# Autodesk Inventor assembly: Assembly1
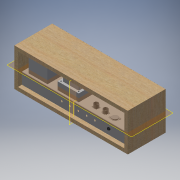
[picture p0: Inventor's stored thumbnail of the model, 180x180]
Saved by Autodesk Inventor 2016 (Build 200138000, 138)
## iProperties
Created: 2015-10-14
Part Number: Assembly1
Document SubType Name: Assembly
Designer: jeremyhale
Author: jeremyhale
## Documents named in this file (16)
- \\psf\Home\Documents\Poorhouse\Amps\p0001\Assembly1.iam
- \\psf\Home\Documents\Poorhouse\Amps\p0001\chassis.ipt
- \\psf\Home\Documents\Poorhouse\Amps\p0001\tube socket 8 pin.ipt
- \\psf\Home\Documents\Poorhouse\Amps\p0001\tube socket 9 pin.ipt
- \\psf\Home\Documents\Poorhouse\Amps\p0001\xmfr power.ipt
- \\psf\Home\Documents\Poorhouse\Amps\p0001\xmfr output.ipt
- \\psf\Home\Documents\Inventor\Content Center Files\R2016\en-US\AS 1427(08)\AS 1427 - M3 x 5(6) I.ipt
- \\psf\Home\Documents\Inventor\Content Center Files\R2016\en-US\AS 1474(1)\AS 1474 - M2.5(1).ipt
- \\psf\Home\Documents\Inventor\Content Center Files\R2016\en-US\AS 1474(1)\AS 1474 - M3.5(1).ipt
- \\psf\Home\Documents\Inventor\Content Center Files\R2016\en-US\AS 1474(1)\AS 1474 - M3(1).ipt
- \\psf\Home\Documents\Poorhouse\Amps\p0001\cabinet.ipt
- \\psf\Home\Documents\Poorhouse\Amps\p0001\iec320_703W-00_04.ipt
- \\psf\Home\Documents\Inventor\Content Center Files\R2016\en-US\AS 1427(07)\AS 1427 - M3 x 10(6) II.ipt
- \\psf\Home\Downloads\switch-toggle.snapshot.2\Toggle_Large_A\Toggle Large A.ipt
- \\psf\Home\Downloads\audio-jack-model-2-1.snapshot.2\AUDIO JACK 2.ipt
- \\psf\Home\Downloads\audio-jack-model-2-1.snapshot.2\AUDIO JACK 2_CPY.ipt
## Components (58 placed, 15 different names)
1. chassis:1 — Rotational:1, Rotational:2, Rotational:3, Rotational:4, Rotational:5, Rotational:6, Rotational:7, Rotational:8, Rotational:9, Rotational:10, Mate:4, Insert:20, Insert:21, Insert:22, Insert:23, Insert:24, Insert:25, Insert:26, Insert:27, Insert:28, Insert:29, Insert:30, Insert:31, Insert:32, Insert:33, Insert:34, Insert:35, Insert:36, Insert:37, Flush:1, Mate:5, Flush:2, Rotational:11, Rotational:12, Mate:11, Mate:13, Rigid:14, Rigid:15, Rigid:16
2. tube socket 8 pin:7 — Rotational:3, Rotational:4, Insert:13, Insert:14
3. xmfr power:1 — Rotational:7, Rotational:8
4. xmfr output:1 — Rotational:9, Rotational:10
5. cabinet:1 — Flush:1, Mate:5, Flush:2
6. iec320_703W-00_04:1 — Rotational:11, Rotational:12, Mate:6, Mate:7
7. AS 1427 Z - Metric M3 x 10:2 — Mate:6, Mate:10
8. AS 1427 Z - Metric M3 x 10:1 — Mate:7, Mate:12
9. AS 1474 - Metric M3:5 — Mate:10, Mate:11
10. AS 1474 - Metric M3:6 — Mate:12, Mate:13
11. Toggle Large A:1 — Rigid:14
12. AUDIO JACK 2:1 — Rigid:15
13. AUDIO JACK 2_CPY:1 — Rigid:16
14. AS 1427 Z - Metric M3 x 5:1 — Insert:1, Mate:3
15. AS 1427 Z - Metric M3 x 5:2 — Insert:2
16. AS 1427 Z - Metric M3 x 5:3 — Insert:3
17. AS 1427 Z - Metric M3 x 5:4 — Insert:4
18. AS 1427 Z - Metric M3 x 5:5 — Insert:5
19. AS 1427 Z - Metric M3 x 5:6 — Insert:6
20. AS 1427 Z - Metric M3 x 5:7 — Insert:7
21. AS 1427 Z - Metric M3 x 5:8 — Insert:8
22. AS 1427 Z - Metric M3 x 5:9 — Insert:9
23. AS 1427 Z - Metric M3 x 5:10 — Insert:10
24. AS 1427 Z - Metric M3 x 5:11 — Insert:11
25. AS 1427 Z - Metric M3 x 5:12 — Insert:12
26. AS 1427 Z - Metric M3 x 5:13 — Insert:13
27. AS 1427 Z - Metric M3 x 5:14 — Insert:14
28. AS 1427 Z - Metric M3 x 5:15 — Insert:15
29. AS 1427 Z - Metric M3 x 5:16 — Insert:16
30. AS 1427 Z - Metric M3 x 5:17 — Insert:17
31. AS 1427 Z - Metric M3 x 5:18 — Insert:18
32. AS 1474 - Metric M2.5:1 — Mate:3, Mate:4
33. AS 1474 - Metric M3.5:1 — Insert:20
34. AS 1474 - Metric M3.5:2 — Insert:21
35. AS 1474 - Metric M3.5:3 — Insert:22
36. AS 1474 - Metric M3.5:4 — Insert:23
37. AS 1474 - Metric M3.5:5 — Insert:24
38. AS 1474 - Metric M3.5:6 — Insert:25
39. AS 1474 - Metric M3.5:7 — Insert:26
40. AS 1474 - Metric M3.5:8 — Insert:27
41. AS 1474 - Metric M3.5:9 — Insert:28
42. AS 1474 - Metric M3.5:10 — Insert:29
43. AS 1474 - Metric M3.5:11 — Insert:30
44. AS 1474 - Metric M3.5:12 — Insert:31
45. AS 1474 - Metric M3.5:13 — Insert:32
46. AS 1474 - Metric M3.5:14 — Insert:33
47. AS 1474 - Metric M3:1 — Insert:34
48. AS 1474 - Metric M3:2 — Insert:35
49. AS 1474 - Metric M3:3 — Insert:36
50. AS 1474 - Metric M3:4 — Insert:37
51. tube socket 8 pin:1 — Rotational:1, Rotational:2, Insert:1, Insert:2
52. tube socket 8 pin:2 — Insert:3, Insert:4
53. tube socket 8 pin:3 — Insert:5, Insert:6
54. tube socket 8 pin:4 — Insert:7, Insert:8
55. tube socket 8 pin:5 — Insert:15, Insert:16
56. tube socket 8 pin:6 — Insert:17, Insert:18
57. tube socket 9 pin:1 — Rotational:5, Rotational:6, Insert:9, Insert:10
58. tube socket 9 pin:2 — Insert:11, Insert:12
## Component patterns: Big Tube Sockets (6 elements), (2 elements, first: tube socket 9 pin:1)
## Relationships (62: Insert 36, RevoluteJoint 12, Mate 9, WeldJoint 3, Flush 2)
- Rotational:1 [RevoluteJoint]: chassis:1 ↔ tube socket 8 pin:1
- Rotational:2 [RevoluteJoint]: chassis:1 ↔ tube socket 8 pin:1
- Rotational:3 [RevoluteJoint]: chassis:1 ↔ tube socket 8 pin:7
- Rotational:4 [RevoluteJoint]: chassis:1 ↔ tube socket 8 pin:7
- Rotational:5 [RevoluteJoint]: chassis:1 ↔ tube socket 9 pin:1
- Rotational:6 [RevoluteJoint]: chassis:1 ↔ tube socket 9 pin:1
- Rotational:7 [RevoluteJoint]: chassis:1 ↔ xmfr power:1
- Rotational:8 [RevoluteJoint]: chassis:1 ↔ xmfr power:1
- Rotational:9 [RevoluteJoint]: chassis:1 ↔ xmfr output:1
- Rotational:10 [RevoluteJoint]: chassis:1 ↔ xmfr output:1
- Insert:1: AS 1427 Z - Metric M3 x 5:1 ↔ tube socket 8 pin:1
- Insert:2: AS 1427 Z - Metric M3 x 5:2 ↔ tube socket 8 pin:1
- Insert:3: AS 1427 Z - Metric M3 x 5:3 ↔ tube socket 8 pin:2
- Insert:4: AS 1427 Z - Metric M3 x 5:4 ↔ tube socket 8 pin:2
- Insert:5: AS 1427 Z - Metric M3 x 5:5 ↔ tube socket 8 pin:3
- Insert:6: AS 1427 Z - Metric M3 x 5:6 ↔ tube socket 8 pin:3
- Insert:7: AS 1427 Z - Metric M3 x 5:7 ↔ tube socket 8 pin:4
- Insert:8: AS 1427 Z - Metric M3 x 5:8 ↔ tube socket 8 pin:4
- Insert:9: AS 1427 Z - Metric M3 x 5:9 ↔ tube socket 9 pin:1
- Insert:10: AS 1427 Z - Metric M3 x 5:10 ↔ tube socket 9 pin:1
- Insert:11: AS 1427 Z - Metric M3 x 5:11 ↔ tube socket 9 pin:2
- Insert:12: AS 1427 Z - Metric M3 x 5:12 ↔ tube socket 9 pin:2
- Insert:13: tube socket 8 pin:7 ↔ AS 1427 Z - Metric M3 x 5:13
- Insert:14: tube socket 8 pin:7 ↔ AS 1427 Z - Metric M3 x 5:14
- Insert:15: AS 1427 Z - Metric M3 x 5:15 ↔ tube socket 8 pin:5
- Insert:16: AS 1427 Z - Metric M3 x 5:16 ↔ tube socket 8 pin:5
- Insert:17: AS 1427 Z - Metric M3 x 5:17 ↔ tube socket 8 pin:6
- Insert:18: AS 1427 Z - Metric M3 x 5:18 ↔ tube socket 8 pin:6
- Mate:3: AS 1427 Z - Metric M3 x 5:1 ↔ AS 1474 - Metric M2.5:1
- Mate:4: chassis:1 ↔ AS 1474 - Metric M2.5:1
- Insert:20: chassis:1 ↔ AS 1474 - Metric M3.5:1
- Insert:21: chassis:1 ↔ AS 1474 - Metric M3.5:2
- Insert:22: chassis:1 ↔ AS 1474 - Metric M3.5:3
- Insert:23: chassis:1 ↔ AS 1474 - Metric M3.5:4
- Insert:24: chassis:1 ↔ AS 1474 - Metric M3.5:5
- Insert:25: chassis:1 ↔ AS 1474 - Metric M3.5:6
- Insert:26: chassis:1 ↔ AS 1474 - Metric M3.5:7
- Insert:27: chassis:1 ↔ AS 1474 - Metric M3.5:8
- Insert:28: chassis:1 ↔ AS 1474 - Metric M3.5:9
- Insert:29: chassis:1 ↔ AS 1474 - Metric M3.5:10
- Insert:30: chassis:1 ↔ AS 1474 - Metric M3.5:11
- Insert:31: chassis:1 ↔ AS 1474 - Metric M3.5:12
- Insert:32: chassis:1 ↔ AS 1474 - Metric M3.5:13
- Insert:33: chassis:1 ↔ AS 1474 - Metric M3.5:14
- Insert:34: chassis:1 ↔ AS 1474 - Metric M3:1
- Insert:35: chassis:1 ↔ AS 1474 - Metric M3:2
- Insert:36: chassis:1 ↔ AS 1474 - Metric M3:3
- Insert:37: chassis:1 ↔ AS 1474 - Metric M3:4
- Flush:1: chassis:1 ↔ cabinet:1
- Mate:5: chassis:1 ↔ cabinet:1
- Flush:2 (-19.05 mm): chassis:1 ↔ cabinet:1
- Rotational:11 [RevoluteJoint]: chassis:1 ↔ iec320_703W-00_04:1
- Rotational:12 [RevoluteJoint]: chassis:1 ↔ iec320_703W-00_04:1
- Mate:6: iec320_703W-00_04:1 ↔ AS 1427 Z - Metric M3 x 10:2
- Mate:7: iec320_703W-00_04:1 ↔ AS 1427 Z - Metric M3 x 10:1
- Mate:10: AS 1427 Z - Metric M3 x 10:2 ↔ AS 1474 - Metric M3:5
- Mate:11: chassis:1 ↔ AS 1474 - Metric M3:5
- Mate:12: AS 1427 Z - Metric M3 x 10:1 ↔ AS 1474 - Metric M3:6
- Mate:13: chassis:1 ↔ AS 1474 - Metric M3:6
- Rigid:14 [WeldJoint]: chassis:1 ↔ Toggle Large A:1
- Rigid:15 [WeldJoint]: chassis:1 ↔ AUDIO JACK 2:1
- Rigid:16 [WeldJoint]: chassis:1 ↔ AUDIO JACK 2_CPY:1
